# Autodesk Inventor assembly: Correct nut unmodified ASSembly
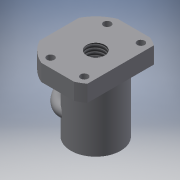
[picture p0: Inventor's stored thumbnail of the model, 180x180]
Saved by Autodesk Inventor 2018 (Build 220112000, 112)
## iProperties
Created: 2017-07-25
Part Number: Correct nut unmodified ASSembly
Document SubType Name: Assembly
Designer: M227562
Author: M227562
## Documents named in this file (3)
- S:\Mechanical_Eng\Fremantle\Joel P\Lathe2018\Lathe with updated parts (LATEST of 20 06 17)\X Axis Nut Correct\Correct nut unmodified ASSembly.iam
- S:\Mechanical_Eng\Fremantle\Joel P\Lathe2018\Lathe with updated parts (LATEST of 20 06 17)\X Axis Nut Correct\Tube for ball screew.ipt
- S:\Mechanical_Eng\Fremantle\Joel P\Lathe2018\Lathe with updated parts (LATEST of 20 06 17)\X Axis Nut Correct\NUT TEST.ipt
## Components (2 placed, 2 different names)
1. Tube for ball screew:1 — Rotational:1
2. NUT TEST:1 — Rotational:1
## Relationships (1: RevoluteJoint 1)
- Rotational:1 [RevoluteJoint] (-1.8 mm): Tube for ball screew:1 ↔ NUT TEST:1
